# Autodesk Inventor assembly: New redesign Assembly
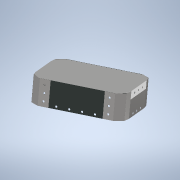
[picture p0: Inventor's stored thumbnail of the model, 180x180]
Saved by Autodesk Inventor 2020 (Build 240168000, 168)
## iProperties
Created: 2022-07-17
Part Number: New redesign Assembly
Document SubType Name: Assembly
Designer: karimi2
Author: karimi2
## Documents named in this file (4)
- C:\Users\karimi2\Documents\PROJECT\src\New redesign Assembly.iam
- C:\Users\karimi2\Documents\PROJECT\src\New front.ipt
- C:\Users\karimi2\Documents\PROJECT\src\New side.ipt
- C:\Users\karimi2\Documents\PROJECT\src\New top.ipt
## Components (5 placed, 3 different names)
1. New front:1 — Mate:1, Mate:2, Mate:3, Mate:9, Mate:10, Mate:11
2. New side:1 — Mate:1, Mate:2, Mate:3, Mate:4, Mate:5, Mate:6
3. New front:2 — Mate:4, Mate:5, Mate:6, Mate:7, Mate:8, Mate:12, Mate:13, Mate:14
4. New side:2 — Mate:7, Mate:8, Mate:9, Mate:10, Mate:11
5. New top:1 — Mate:12, Mate:13, Mate:14
## Relationships (14: Mate 14)
- Mate:1: New front:1 ↔ New side:1
- Mate:2: New front:1 ↔ New side:1
- Mate:3: New front:1 ↔ New side:1
- Mate:4: New side:1 ↔ New front:2
- Mate:5: New side:1 ↔ New front:2
- Mate:6: New side:1 ↔ New front:2
- Mate:7: New front:2 ↔ New side:2
- Mate:8: New front:2 ↔ New side:2
- Mate:9: New front:1 ↔ New side:2
- Mate:10: New front:1 ↔ New side:2
- Mate:11: New front:1 ↔ New side:2
- Mate:12: New front:2 ↔ New top:1
- Mate:13: New front:2 ↔ New top:1
- Mate:14: New front:2 ↔ New top:1
